# Autodesk Inventor assembly: ENSAMBLE_V3
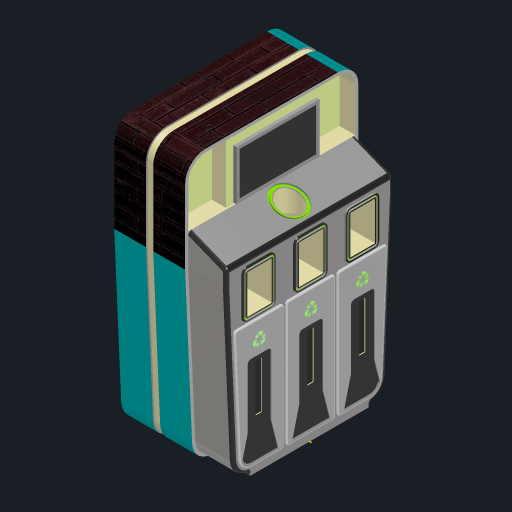
[picture p0: Inventor's stored thumbnail of the model, 512x512]
Saved by Autodesk Inventor 2024.3 (Build 283343000, 343)
## iProperties
Created: 2024-05-12
Part Number: ENSAMBLE_V3
Material: Generic
Document SubType Name: Assembly
Designer: Niler
Author: Niler
## Documents named in this file (3)
- C:\Users\Niler\OneDrive\Escritorio\RECICLADOR\RECICLADOR_MODELO_3D\VERSION_COMPLETA\ENSAMBLE_V3.iam
- C:\Users\Niler\OneDrive\Escritorio\RECICLADOR\RECICLADOR_MODELO_3D\VERSION_COMPLETA\CARCASA_V3.ipt
- C:\Users\Niler\OneDrive\Escritorio\RECICLADOR\RECICLADOR_MODELO_3D\VERSION_COMPLETA\DIMENSIONES_PANTALLA_22.ipt
## Components (2 placed, 2 different names)
1. CARCASA_V3:1 — Mate:1, Flush:1, Flush:2
2. DIMENSIONES_PANTALLA_22:1 — Mate:1, Flush:1, Flush:2
## Relationships (3: Flush 2, Mate 1)
- Mate:1: CARCASA_V3:1 ↔ DIMENSIONES_PANTALLA_22:1
- Flush:1 (-16.5 mm): CARCASA_V3:1 ↔ DIMENSIONES_PANTALLA_22:1
- Flush:2 (50 mm): CARCASA_V3:1 ↔ DIMENSIONES_PANTALLA_22:1
